# Autodesk Inventor assembly: Sestava1
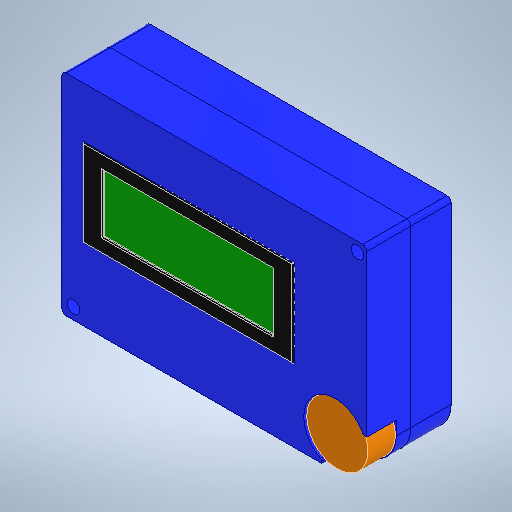
[picture p0: Inventor's stored thumbnail of the model, 512x512]
Saved by Autodesk Inventor 2025.2 (Build 292293000, 293)
## iProperties
Created: 2025-03-25
Part Number: Sestava1
Document SubType Name: Assembly
Designer: jakub
Author: jakub
## Documents named in this file (5)
- C:\Users\jakub\OneDrive\Plocha\Sestava1.iam
- C:\Users\jakub\OneDrive\Plocha\Krabička_horni.ipt
- C:\Users\jakub\OneDrive\Plocha\Krabicka_dolni.ipt
- C:\Users\jakub\OneDrive\Plocha\Tlacitko.ipt
- C:\Users\jakub\OneDrive\Plocha\Součást12.ipt
## Components (5 placed, 4 different names)
1. Krabicka_dolni:1 — Proti sobě:1, Proti sobě:2
2. Krabička_horni:1 — Proti sobě:1, Proti sobě:2, Proti sobě:3, Proti sobě:4, Proti sobě:5, Proti sobě:6, Proti sobě:7, Proti sobě:8
3. Tlacitko:1 — Proti sobě:3, Proti sobě:4
4. Tlacitko:2 — Proti sobě:5, Proti sobě:6
5. Součást12:1 — Proti sobě:7, Proti sobě:8
## Relationships (8: Mate 8)
- Proti sobě:1 [Mate]: Krabicka_dolni:1 ↔ Krabička_horni:1
- Proti sobě:2 [Mate]: Krabicka_dolni:1 ↔ Krabička_horni:1
- Proti sobě:3 [Mate]: Krabička_horni:1 ↔ Tlacitko:1
- Proti sobě:4 [Mate]: Krabička_horni:1 ↔ Tlacitko:1
- Proti sobě:5 [Mate]: Krabička_horni:1 ↔ Tlacitko:2
- Proti sobě:6 [Mate]: Krabička_horni:1 ↔ Tlacitko:2
- Proti sobě:7 [Mate]: Krabička_horni:1 ↔ Součást12:1
- Proti sobě:8 [Mate]: Krabička_horni:1 ↔ Součást12:1
